# Autodesk Inventor assembly: Front Crossbrace
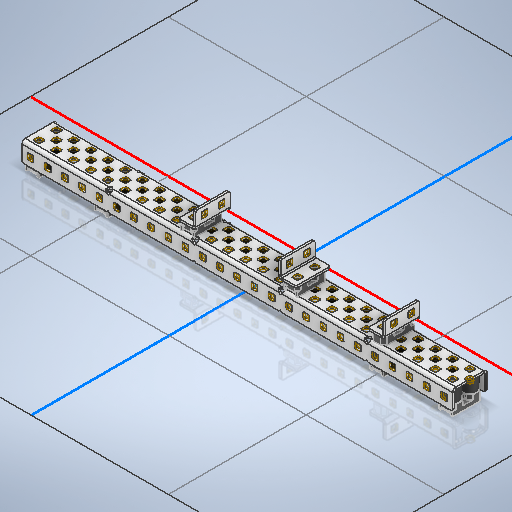
[picture p0: Inventor's stored thumbnail of the model, 512x512]
Saved by Autodesk Inventor 2026 (Build 300175000, 175)
## iProperties
Created: 2025-04-02
Part Number: Front Crossbrace
Document SubType Name: Assembly
Designer: avere
Author: avere
## Documents named in this file (8)
- C:\Users\avere\OneDrive\Documents\VEX-CAD\V5-CAD\drivetrain\Braces\Front Crossbrace.iam
- C:\Users\avere\OneDrive\Documents\VEX-CAD\VEX-CAD-Inventor\Structure\C Channel\Aluminum 1x2x1\Alu C 1x2x1x25.ipt
- C:\Users\avere\OneDrive\Documents\VEX-CAD\VEX-CAD-Inventor\Structure\Angle\Aluminum 1x1\Alu Angle 1x1x2.ipt
- C:\Users\avere\OneDrive\Documents\VEX-CAD\VEX-CAD-Inventor\Motion\Shaft LS\Bearing Flat - Cut.ipt
- C:\Users\avere\OneDrive\Documents\VEX-CAD\VEX-CAD-Inventor\Motion\Spacers\Spacer Nylon .375 OD\NSpacer .375 OD x .375.ipt
- C:\Users\avere\OneDrive\Documents\VEX-CAD\VEX-CAD-Inventor\Motion\Spacers\Spacer Nylon .375 OD.ipt
- C:\Users\avere\OneDrive\Documents\VEX-CAD\VEX-CAD-Inventor\Motion\Spacers\Washer Steel\SWasher .375 OD x .062500.ipt
- C:\Users\avere\OneDrive\Documents\VEX-CAD\VEX-CAD-Inventor\Motion\Spacers\Washer Steel.ipt
## Components (27 placed, 5 different names)
1. Alu C 1x2x1x25:1 — Mate:1, Mate:2, Mate:3, Insert:1, Mate:4, Insert:2, Mate:5, Insert:3, Insert:4, Insert:9, Mate:8, Insert:10, Mate:10
2. Alu Angle 1x1x2:1 — Insert:1, Mate:4, Mate:6
3. Alu Angle 1x1x2:2 — Insert:2, Mate:5, Mate:7
4. Bearing Flat - Cut:1 — Insert:3, Mate:6
5. Bearing Flat - Cut:2 — Insert:4, Mate:7
6. Alu Angle 1x1x2:3 — Insert:11
7. Bearing Flat - Cut:8 — Insert:10, Mate:10, Insert:11
8. Bearing Flat - Cut:4 — Insert:6, Insert:8, Mate:8
9. NSpacer .375 OD x .375:1 — Insert:5, Insert:6
10. SWasher .375 OD x .062500:1 — Insert:5, Insert:9
11. NSpacer .375 OD x .375:2 — Insert:8
12. SWasher .375 OD x .062500:2
13. Bearing Flat - Cut:5
14. NSpacer .375 OD x .375:3
15. SWasher .375 OD x .062500:3
16. NSpacer .375 OD x .375:4
17. SWasher .375 OD x .062500:4
18. Bearing Flat - Cut:6
19. NSpacer .375 OD x .375:5
20. SWasher .375 OD x .062500:5
21. NSpacer .375 OD x .375:6
22. SWasher .375 OD x .062500:6
23. Bearing Flat - Cut:7
24. NSpacer .375 OD x .375:7
25. SWasher .375 OD x .062500:7
26. NSpacer .375 OD x .375:8
27. SWasher .375 OD x .062500:8
## Component patterns: (4 elements, first: Bearing Flat - Cut:4 + NSpacer .375 OD x .375:1 + SWasher .375 OD x .062500:1 + NSpacer .375 OD x .375:2 + SWasher .375 OD x .062500:2)
## Relationships (21: Insert 11, Mate 10)
- Mate:1 (25.4 mm): Alu C 1x2x1x25:1
- Mate:2 (-158.75 mm): Alu C 1x2x1x25:1
- Mate:3 (50.8 mm): Alu C 1x2x1x25:1
- Insert:1 (6.35 mm): Alu C 1x2x1x25:1 ↔ Alu Angle 1x1x2:1
- Mate:4: Alu C 1x2x1x25:1 ↔ Alu Angle 1x1x2:1
- Insert:2 (6.35 mm): Alu C 1x2x1x25:1 ↔ Alu Angle 1x1x2:2
- Mate:5: Alu C 1x2x1x25:1 ↔ Alu Angle 1x1x2:2
- Insert:3: Alu C 1x2x1x25:1 ↔ Bearing Flat - Cut:1
- Mate:6: Alu Angle 1x1x2:1 ↔ Bearing Flat - Cut:1
- Insert:4: Alu C 1x2x1x25:1 ↔ Bearing Flat - Cut:2
- Mate:7: Alu Angle 1x1x2:2 ↔ Bearing Flat - Cut:2
- Insert:5: NSpacer .375 OD x .375:1 ↔ SWasher .375 OD x .062500:1
- Insert:6: Bearing Flat - Cut:4 ↔ NSpacer .375 OD x .375:1
- [Insert]: NSpacer .375 OD x .375:2 ↔ SWasher .375 OD x .062500:2
- Insert:8: Bearing Flat - Cut:4 ↔ NSpacer .375 OD x .375:2
- Insert:9: Alu C 1x2x1x25:1 ↔ SWasher .375 OD x .062500:1
- Mate:8: Alu C 1x2x1x25:1 ↔ Bearing Flat - Cut:4
- [Mate]: Alu Angle 1x1x2:3 ↔ Bearing Flat - Cut:8
- Insert:10: Alu C 1x2x1x25:1 ↔ Bearing Flat - Cut:8
- Mate:10: Alu C 1x2x1x25:1 ↔ Bearing Flat - Cut:8
- Insert:11: Alu Angle 1x1x2:3 ↔ Bearing Flat - Cut:8
## Named parameters: d13_d11 = 0 mm, d21_d8 = 0 mm
